# Autodesk Inventor assembly: 14in slide
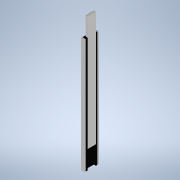
[picture p0: Inventor's stored thumbnail of the model, 180x180]
Saved by Autodesk Inventor 2020.1 (Build 241239000, 239)
## iProperties
Created: 2019-09-13
Part Number: 14in slide
Document SubType Name: Assembly
Designer: alpha
Author: alpha
## Documents named in this file (4)
- C:\Users\tbloo\Documents\GitHub\AO_Robotics\CAD\Projects\Timothy Bloot\14in slide.iam
- C:\Users\tbloo\Documents\GitHub\AO_Robotics\CAD\Projects\Timothy Bloot\14in-slide-pt_1.ipt
- C:\Users\tbloo\Documents\GitHub\AO_Robotics\CAD\Projects\Timothy Bloot\14in-slide-pt_2.ipt
- C:\Users\tbloo\Documents\GitHub\AO_Robotics\CAD\Projects\Timothy Bloot\14in-slide-pt_3.ipt
## Components (3 placed, 3 different names)
1. 14in-slide-pt_1:1 — Slider:1
2. 14in-slide-pt_2:1 — Slider:1, Slider:2
3. 14in-slide-pt_3:1 — Slider:2
## Relationships (2: TranslationJoint 2)
- Slider:1 [TranslationJoint]: 14in-slide-pt_1:1 ↔ 14in-slide-pt_2:1
- Slider:2 [TranslationJoint]: 14in-slide-pt_2:1 ↔ 14in-slide-pt_3:1
